# Autodesk Inventor assembly: tower
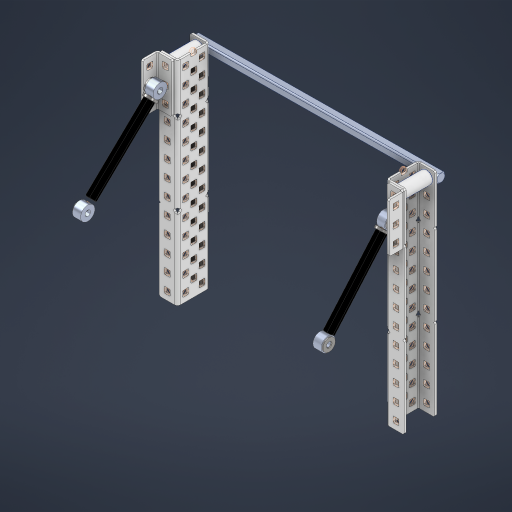
[picture p0: Inventor's stored thumbnail of the model, 512x512]
Saved by Autodesk Inventor 2024 (Build 280153000, 153)
## iProperties
Created: 2023-10-19
Part Number: tower
Document SubType Name: Assembly
Designer: avere
Author: avere
## Documents named in this file (6)
- D:\vex_robotics\hardware\cad\goated_v0.1\catapult\tower.iam
- D:\vex_robotics\hardware\cad\VEX-CAD-Inventor-1.41\Structure\C Channel\Aluminum 1x2x1\Alu C 1x2x1x13.ipt
- D:\vex_robotics\hardware\cad\hardware\.375 OD Aluminum Spacer 0.875.ipt
- D:\vex_robotics\hardware\cad\VEX-CAD-Inventor-1.41\Structure\Angle\Aluminum 1x1\Alu Angle 1x1x3.ipt
- D:\vex_robotics\hardware\cad\goated_v0.1\catapult\standoff_bracce.iam
- D:\vex_robotics\hardware\cad\goated_v0.1\catapult\custom_parts\hs_hardstop.ipt
## Components (10 placed, 5 different names)
1. Alu C 1x2x1x13:1 — Insert:1, Mate:1, Insert:4, Insert:6, Mate:4, Insert:10
2. Alu C 1x2x1x13:3 — Insert:1, Mate:1
3. .375 OD Aluminum Spacer 0.875:1 — Insert:4
4. Alu Angle 1x1x3:1 — Insert:6, Mate:4, Insert:8
5. Alu Angle 1x1x3:2 — Insert:9, Insert:12, Mate:5
6. standoff_bracce:1 [sub-assembly] — Insert:8
7. standoff_bracce:2 [sub-assembly] — Insert:9
8. hs_hardstop:1 — Insert:10, Insert:11
9. Alu C 1x2x1x13:4 — Insert:11, Insert:12, Mate:5, Insert:13
10. .375 OD Aluminum Spacer 0.875:3 — Insert:13
## Relationships (12: Insert 9, Mate 3)
- Insert:1: Alu C 1x2x1x13:1 ↔ Alu C 1x2x1x13:3
- Mate:1: Alu C 1x2x1x13:1 ↔ Alu C 1x2x1x13:3
- Insert:4: Alu C 1x2x1x13:1 ↔ .375 OD Aluminum Spacer 0.875:1
- Insert:6: Alu C 1x2x1x13:1 ↔ Alu Angle 1x1x3:1
- Mate:4: Alu C 1x2x1x13:1 ↔ Alu Angle 1x1x3:1
- Insert:8: Alu Angle 1x1x3:1 ↔ standoff_bracce:1
- Insert:9: Alu Angle 1x1x3:2 ↔ standoff_bracce:2
- Insert:10: Alu C 1x2x1x13:1 ↔ hs_hardstop:1
- Insert:11: hs_hardstop:1 ↔ Alu C 1x2x1x13:4
- Insert:12: Alu Angle 1x1x3:2 ↔ Alu C 1x2x1x13:4
- Mate:5: Alu Angle 1x1x3:2 ↔ Alu C 1x2x1x13:4
- Insert:13: Alu C 1x2x1x13:4 ↔ .375 OD Aluminum Spacer 0.875:3
